# Autodesk Inventor assembly: MicroUSB Breakout
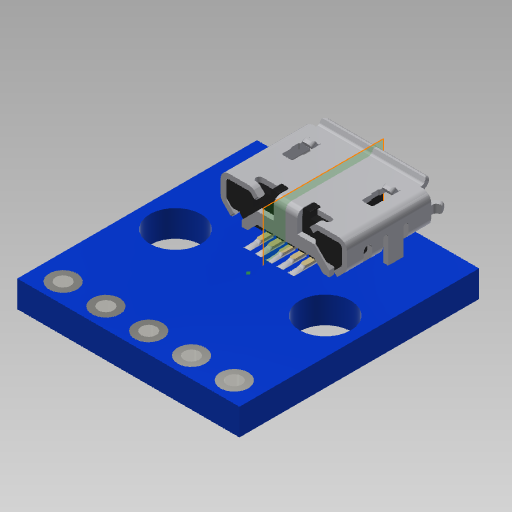
[picture p0: Inventor's stored thumbnail of the model, 512x512]
Saved by Autodesk Inventor 2020 (Build 240168000, 168)
## iProperties
Created: 2018-07-27
Part Number: MicroUSB Breakout
Document SubType Name: Assembly
Designer: amsmi
Author: amsmi
## Documents named in this file (3)
- C:\Users\Alex\Documents\Inventor Modeling\Legacy\Nanodevelopment Lab\Pirani Gauge\Final Readout\MicroUSB Breakout.iam
- C:\Users\Alex\Documents\Inventor Modeling\Legacy\Nanodevelopment Lab\Pirani Gauge\Final Readout\MicroUSB.iam
- C:\Users\Alex\Documents\Inventor Modeling\Legacy\Nanodevelopment Lab\Pirani Gauge\Final Readout\pcb_microusb.ipt
## Components (2 placed, 2 different names)
1. MicroUSB:1 [sub-assembly] — Mate:5
2. pcb_microusb:1
## Relationships (7: Mate 5, Angle 1, Flush 1)
- [Mate]: pcb_microusb:1
- [Mate]: pcb_microusb:1
- [Mate]: pcb_microusb:1
- [Mate]: MicroUSB:1 ↔ pcb_microusb:1
- [Angle] (0 deg): MicroUSB:1 ↔ pcb_microusb:1
- Mate:5: MicroUSB:1
- [Flush]: MicroUSB:1 ↔ pcb_microusb:1
